# Autodesk Inventor assembly: ABD_Slider_Set_v2_2025
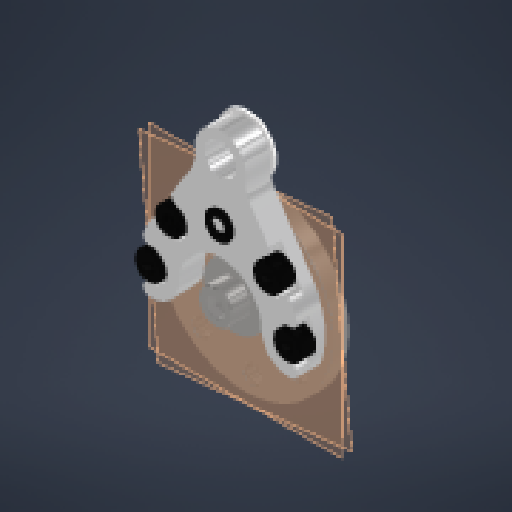
[picture p0: Inventor's stored thumbnail of the model, 512x512]
Saved by Autodesk Inventor 2024.3 (Build 283343000, 343)
## iProperties
Created: 2025-01-09
Part Number: ABD_Slider_Set_v2_2025
Document SubType Name: Assembly
Designer: ASUS
Author: ASUS
## Documents named in this file (6)
- C:\Users\ASUS\Desktop\Anti_Backlash_Structure_OP\V2_Frame(2025)\ABD_Slider_Set_v2_2025.iam
- C:\Users\ASUS\Desktop\2024_Robit_Hardware\ROBOCUP_2024_eindhoven\부품\ROBOTIS(Inventor 2023 ver.)\혼\64-106Horn.ipt
- C:\Users\ASUS\Desktop\Anti_Backlash_Structure_OP\MISUMI\CSH-STN-M3-10_203.ipt
- C:\Users\ASUS\Desktop\Anti_Backlash_Structure_OP\MISUMI\4mm_ABD_set.iam
- C:\Users\ASUS\Desktop\Anti_Backlash_Structure_OP\MISUMI\TT-0409-051.ipt
- C:\Users\ASUS\Desktop\Anti_Backlash_Structure_OP\V2_Frame(2025)\Slider_crank_horn_v2_2025.ipt
## Components (5 placed, 5 different names)
1. 64-106Horn:1
2. CSH-STN-M3-10_203:1
3. 4mm_ABD_set:1 [sub-assembly]
4. Slider_crank_horn_v2_2025:1 — 삽입:5
5. TT-0409-051:1 — 삽입:5
## Relationships (5: Insert 4, Mate 1)
- [Insert]: 64-106Horn:1 ↔ CSH-STN-M3-10_203:1
- [Insert]: 64-106Horn:1 ↔ Slider_crank_horn_v2_2025:1
- [Insert]: 4mm_ABD_set:1 ↔ Slider_crank_horn_v2_2025:1
- [Mate]: 4mm_ABD_set:1 ↔ Slider_crank_horn_v2_2025:1
- 삽입:5 [Insert]: Slider_crank_horn_v2_2025:1 ↔ TT-0409-051:1
